# Autodesk Inventor assembly: Tracking Wheel Assembly
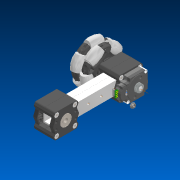
[picture p0: Inventor's stored thumbnail of the model, 180x180]
Saved by Autodesk Inventor 2022.2 (Build 262287000, 287)
## iProperties
Created: 2022-01-04
Part Number: Tracking Wheel Assembly
Document SubType Name: Assembly
Designer: omard
Mass: 324.916 g
Surface Area: 2107.74 cm^2
Volume: 267.656 cm^3
Density: 1.21393 g/cm^3
Author: omard
## Documents named in this file (12)
- D:\omard\OneDrive - Auburn University\BasketBall Shooting Robot\Tracking Wheel Assembly.iam
- D:\omard\OneDrive - Auburn University\BasketBall Shooting Robot\VEX Parts\302 (1_4 ThunderSquare) ID x 0.875 OD x 0.280 WD (Flanged Bearing) (217-5830) .ipt
- D:\omard\OneDrive - Auburn University\BasketBall Shooting Robot\VEX Parts\VersaBlock Mini Kit (217-5852).iam
- D:\omard\OneDrive - Auburn University\BasketBall Shooting Robot\VEX Parts\V5 Rotation Sensor (276-6050).iam
- D:\omard\OneDrive - Auburn University\BasketBall Shooting Robot\VEX Parts\3.25 Omni-Directional Wheel (217-4775).iam
- D:\omard\OneDrive - Auburn University\BasketBall Shooting Robot\VEX Parts\1_2 VersaHex Adapters (1_4 Square Bore, 1_4 Long) (6 Pack) (217-5950).ipt
- D:\omard\OneDrive - Auburn University\BasketBall Shooting Robot\VEX Parts\Low Profile High Strength Clamping Shaft Collar (276-7580).ipt
- D:\omard\OneDrive - Auburn University\BasketBall Shooting Robot\VEX Parts\Special Cut\1 x 1 x 0.100 x 6 Tracking Wheel Pre-Drilled VersaFrame Aluminum Tube Stock Cut (217-4104).ipt
- D:\omard\OneDrive - Auburn University\BasketBall Shooting Robot\VEX Parts\4.4 High Strength Shaft Cut (276-3524).ipt
- D:\omard\OneDrive - Auburn University\BasketBall Shooting Robot\VEX Parts\#8-32 Nylock Nut (275-1027).ipt
- D:\omard\OneDrive - Auburn University\BasketBall Shooting Robot\VEX Parts\VersaPlanetary Integrated Encoder (217-5046).iam
- D:\omard\OneDrive - Auburn University\BasketBall Shooting Robot\Versa Encoder Adapter.ipt
## Components (18 placed, 11 different names)
1. 302 (1_4 ThunderSquare) ID x 0.875 OD x 0.280 WD (Flanged Bearing) (217-5830) :1 — Mate:1, Mate:4, Angle:1, Mate:9, Mate:11
2. 302 (1_4 ThunderSquare) ID x 0.875 OD x 0.280 WD (Flanged Bearing) (217-5830) :2 — Mate:2, Mate:3, Angle:2, Mate:22, Mate:23, Mate:25
3. VersaBlock Mini Kit (217-5852):1 [sub-assembly] — Mate:1, Mate:2, Mate:3, Mate:4, Angle:1, Angle:2, Angle:5, Flush:1, Flush:2, Mate:12, Mate:13, Mate:27, Mate:31
4. 302 (1_4 ThunderSquare) ID x 0.875 OD x 0.280 WD (Flanged Bearing) (217-5830) :3 — Mate:10
5. 302 (1_4 ThunderSquare) ID x 0.875 OD x 0.280 WD (Flanged Bearing) (217-5830) :4
6. VersaBlock Mini Kit (217-5852):2 [sub-assembly] — Flush:2, Angle:6, Angle:13
7. 1 x 1 x 0.100 x 6 Tracking Wheel Pre-Drilled VersaFrame Aluminum Tube Stock Cut (217-4104):1 — Mate:9, Angle:5, Flush:1, Mate:10, Angle:6, Mate:24, Angle:13, Angle:16
8. V5 Rotation Sensor (276-6050):1 [sub-assembly] — Mate:11, Mate:12, Mate:13, Angle:11, Angle:12, Mate:26, Angle:14, Mate:27, Mate:28, Mate:29, Angle:15
9. 3.25 Omni-Directional Wheel (217-4775):1 [sub-assembly] — Angle:7, Mate:14, Mate:15, Mate:16, Mate:17
10. 1_2 VersaHex Adapters (1_4 Square Bore, 1_4 Long) (6 Pack) (217-5950):1 — Angle:8, Mate:16, Mate:17, Angle:10, Mate:19, Mate:20
11. 1_2 VersaHex Adapters (1_4 Square Bore, 1_4 Long) (6 Pack) (217-5950):2 — Angle:7, Mate:14, Mate:15, Angle:8, Mate:18, Angle:9, Mate:21
12. Low Profile High Strength Clamping Shaft Collar (276-7580):1 — Angle:10, Mate:19, Mate:20, Angle:11, Flush:3
13. Low Profile High Strength Clamping Shaft Collar (276-7580):2 — Mate:18, Angle:9, Mate:21, Mate:22, Mate:23
14. Low Profile High Strength Clamping Shaft Collar (276-7580):3 — Angle:12, Mate:24, Mate:25
15. 4.4 High Strength Shaft Cut (276-3524):1 — Mate:26, Angle:14, Flush:3, Mate:30, Mate:32
16. #8-32 Nylock Nut (275-1027):1 — Mate:28, Mate:29, Angle:15
17. VersaPlanetary Integrated Encoder (217-5046):1 [sub-assembly] — Mate:30, Angle:16, Mate:31, Mate:33
18. Versa Encoder Adapter:1 — Mate:32, Mate:33
## Relationships (52: Mate 33, Angle 16, Flush 3)
- Mate:1: 302 (1_4 ThunderSquare) ID x 0.875 OD x 0.280 WD (Flanged Bearing) (217-5830) :1 ↔ VersaBlock Mini Kit (217-5852):1
- Mate:2: 302 (1_4 ThunderSquare) ID x 0.875 OD x 0.280 WD (Flanged Bearing) (217-5830) :2 ↔ VersaBlock Mini Kit (217-5852):1
- Mate:3: 302 (1_4 ThunderSquare) ID x 0.875 OD x 0.280 WD (Flanged Bearing) (217-5830) :2 ↔ VersaBlock Mini Kit (217-5852):1
- Mate:4: 302 (1_4 ThunderSquare) ID x 0.875 OD x 0.280 WD (Flanged Bearing) (217-5830) :1 ↔ VersaBlock Mini Kit (217-5852):1
- Angle:1 (0 deg): 302 (1_4 ThunderSquare) ID x 0.875 OD x 0.280 WD (Flanged Bearing) (217-5830) :1 ↔ VersaBlock Mini Kit (217-5852):1
- Angle:2 (0 deg): 302 (1_4 ThunderSquare) ID x 0.875 OD x 0.280 WD (Flanged Bearing) (217-5830) :2 ↔ VersaBlock Mini Kit (217-5852):1
- [Mate]: 302 (1_4 ThunderSquare) ID x 0.875 OD x 0.280 WD (Flanged Bearing) (217-5830) :3 ↔ VersaBlock Mini Kit (217-5852):2
- [Mate]: 302 (1_4 ThunderSquare) ID x 0.875 OD x 0.280 WD (Flanged Bearing) (217-5830) :4 ↔ VersaBlock Mini Kit (217-5852):2
- [Mate]: 302 (1_4 ThunderSquare) ID x 0.875 OD x 0.280 WD (Flanged Bearing) (217-5830) :4 ↔ VersaBlock Mini Kit (217-5852):2
- [Mate]: 302 (1_4 ThunderSquare) ID x 0.875 OD x 0.280 WD (Flanged Bearing) (217-5830) :3 ↔ VersaBlock Mini Kit (217-5852):2
- [Angle] (0 deg): 302 (1_4 ThunderSquare) ID x 0.875 OD x 0.280 WD (Flanged Bearing) (217-5830) :3 ↔ VersaBlock Mini Kit (217-5852):2
- [Angle] (0 deg): 302 (1_4 ThunderSquare) ID x 0.875 OD x 0.280 WD (Flanged Bearing) (217-5830) :4 ↔ VersaBlock Mini Kit (217-5852):2
- Mate:9: 302 (1_4 ThunderSquare) ID x 0.875 OD x 0.280 WD (Flanged Bearing) (217-5830) :1 ↔ 1 x 1 x 0.100 x 6 Tracking Wheel Pre-Drilled VersaFrame Aluminum Tube Stock Cut (217-4104):1
- Angle:5 (0 deg): VersaBlock Mini Kit (217-5852):1 ↔ 1 x 1 x 0.100 x 6 Tracking Wheel Pre-Drilled VersaFrame Aluminum Tube Stock Cut (217-4104):1
- Flush:1: VersaBlock Mini Kit (217-5852):1 ↔ 1 x 1 x 0.100 x 6 Tracking Wheel Pre-Drilled VersaFrame Aluminum Tube Stock Cut (217-4104):1
- Mate:10: 302 (1_4 ThunderSquare) ID x 0.875 OD x 0.280 WD (Flanged Bearing) (217-5830) :3 ↔ 1 x 1 x 0.100 x 6 Tracking Wheel Pre-Drilled VersaFrame Aluminum Tube Stock Cut (217-4104):1
- Flush:2: VersaBlock Mini Kit (217-5852):1 ↔ VersaBlock Mini Kit (217-5852):2
- Angle:6 (0 deg): VersaBlock Mini Kit (217-5852):2 ↔ 1 x 1 x 0.100 x 6 Tracking Wheel Pre-Drilled VersaFrame Aluminum Tube Stock Cut (217-4104):1
- Mate:11: 302 (1_4 ThunderSquare) ID x 0.875 OD x 0.280 WD (Flanged Bearing) (217-5830) :1 ↔ V5 Rotation Sensor (276-6050):1
- Mate:12: VersaBlock Mini Kit (217-5852):1 ↔ V5 Rotation Sensor (276-6050):1
- Mate:13: VersaBlock Mini Kit (217-5852):1 ↔ V5 Rotation Sensor (276-6050):1
- Angle:7 (0 deg): 3.25 Omni-Directional Wheel (217-4775):1 ↔ 1_2 VersaHex Adapters (1_4 Square Bore, 1_4 Long) (6 Pack) (217-5950):2
- Mate:14: 3.25 Omni-Directional Wheel (217-4775):1 ↔ 1_2 VersaHex Adapters (1_4 Square Bore, 1_4 Long) (6 Pack) (217-5950):2
- Mate:15: 3.25 Omni-Directional Wheel (217-4775):1 ↔ 1_2 VersaHex Adapters (1_4 Square Bore, 1_4 Long) (6 Pack) (217-5950):2
- Angle:8 (0 deg): 1_2 VersaHex Adapters (1_4 Square Bore, 1_4 Long) (6 Pack) (217-5950):1 ↔ 1_2 VersaHex Adapters (1_4 Square Bore, 1_4 Long) (6 Pack) (217-5950):2
- Mate:16: 3.25 Omni-Directional Wheel (217-4775):1 ↔ 1_2 VersaHex Adapters (1_4 Square Bore, 1_4 Long) (6 Pack) (217-5950):1
- Mate:17: 3.25 Omni-Directional Wheel (217-4775):1 ↔ 1_2 VersaHex Adapters (1_4 Square Bore, 1_4 Long) (6 Pack) (217-5950):1
- Mate:18: 1_2 VersaHex Adapters (1_4 Square Bore, 1_4 Long) (6 Pack) (217-5950):2 ↔ Low Profile High Strength Clamping Shaft Collar (276-7580):2
- Angle:9 (0 deg): 1_2 VersaHex Adapters (1_4 Square Bore, 1_4 Long) (6 Pack) (217-5950):2 ↔ Low Profile High Strength Clamping Shaft Collar (276-7580):2
- Angle:10 (0 deg): 1_2 VersaHex Adapters (1_4 Square Bore, 1_4 Long) (6 Pack) (217-5950):1 ↔ Low Profile High Strength Clamping Shaft Collar (276-7580):1
- Mate:19: 1_2 VersaHex Adapters (1_4 Square Bore, 1_4 Long) (6 Pack) (217-5950):1 ↔ Low Profile High Strength Clamping Shaft Collar (276-7580):1
- Mate:20: 1_2 VersaHex Adapters (1_4 Square Bore, 1_4 Long) (6 Pack) (217-5950):1 ↔ Low Profile High Strength Clamping Shaft Collar (276-7580):1
- Mate:21: 1_2 VersaHex Adapters (1_4 Square Bore, 1_4 Long) (6 Pack) (217-5950):2 ↔ Low Profile High Strength Clamping Shaft Collar (276-7580):2
- Mate:22: 302 (1_4 ThunderSquare) ID x 0.875 OD x 0.280 WD (Flanged Bearing) (217-5830) :2 ↔ Low Profile High Strength Clamping Shaft Collar (276-7580):2
- Mate:23: 302 (1_4 ThunderSquare) ID x 0.875 OD x 0.280 WD (Flanged Bearing) (217-5830) :2 ↔ Low Profile High Strength Clamping Shaft Collar (276-7580):2
- Angle:11 (0 deg): V5 Rotation Sensor (276-6050):1 ↔ Low Profile High Strength Clamping Shaft Collar (276-7580):1
- Angle:12 (0 deg): V5 Rotation Sensor (276-6050):1 ↔ Low Profile High Strength Clamping Shaft Collar (276-7580):3
- Mate:24: 1 x 1 x 0.100 x 6 Tracking Wheel Pre-Drilled VersaFrame Aluminum Tube Stock Cut (217-4104):1 ↔ Low Profile High Strength Clamping Shaft Collar (276-7580):3
- Angle:13 (0 deg): VersaBlock Mini Kit (217-5852):2 ↔ 1 x 1 x 0.100 x 6 Tracking Wheel Pre-Drilled VersaFrame Aluminum Tube Stock Cut (217-4104):1
- Mate:25: 302 (1_4 ThunderSquare) ID x 0.875 OD x 0.280 WD (Flanged Bearing) (217-5830) :2 ↔ Low Profile High Strength Clamping Shaft Collar (276-7580):3
- Mate:26: V5 Rotation Sensor (276-6050):1 ↔ 4.4 High Strength Shaft Cut (276-3524):1
- Angle:14 (0 deg): V5 Rotation Sensor (276-6050):1 ↔ 4.4 High Strength Shaft Cut (276-3524):1
- Flush:3: Low Profile High Strength Clamping Shaft Collar (276-7580):1 ↔ 4.4 High Strength Shaft Cut (276-3524):1
- Mate:27: VersaBlock Mini Kit (217-5852):1 ↔ V5 Rotation Sensor (276-6050):1
- Mate:28: V5 Rotation Sensor (276-6050):1 ↔ #8-32 Nylock Nut (275-1027):1
- Mate:29: V5 Rotation Sensor (276-6050):1 ↔ #8-32 Nylock Nut (275-1027):1
- Angle:15 (0 deg): V5 Rotation Sensor (276-6050):1 ↔ #8-32 Nylock Nut (275-1027):1
- Mate:30: 4.4 High Strength Shaft Cut (276-3524):1 ↔ VersaPlanetary Integrated Encoder (217-5046):1
- Angle:16 (0 deg): 1 x 1 x 0.100 x 6 Tracking Wheel Pre-Drilled VersaFrame Aluminum Tube Stock Cut (217-4104):1 ↔ VersaPlanetary Integrated Encoder (217-5046):1
- Mate:31: VersaBlock Mini Kit (217-5852):1 ↔ VersaPlanetary Integrated Encoder (217-5046):1
- Mate:32: 4.4 High Strength Shaft Cut (276-3524):1 ↔ Versa Encoder Adapter:1
- Mate:33: VersaPlanetary Integrated Encoder (217-5046):1 ↔ Versa Encoder Adapter:1
## Named parameters: d7_d0 = 0 mm, d8_d1 = 0 mm, d9_d2 = 0 mm, d10_d4 = 0 mm, d11_d5 = 0 deg, d12_d6 = 0 deg
